# Autodesk Inventor assembly: JIMSCUBE
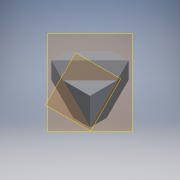
[picture p0: Inventor's stored thumbnail of the model, 180x180]
Saved by Autodesk Inventor 2019 (Build 230136000, 136)
## iProperties
Created: 2019-09-15
Part Number: JIMSCUBE
Document SubType Name: Assembly
Designer: james
Author: james
## Documents named in this file (3)
- F:\JimsDesign\P1001-16bit-CPU\P1001-001 - 16bit CPU\JIMSCUBE.iam
- F:\JimsDesign\P1001-16bit-CPU\P1001-001 - 16bit CPU\JIMSPT.ipt
- F:\JimsDesign\P1001-16bit-CPU\P1001-001 - 16bit CPU\jimscube.ipt
## Components (2 placed, 2 different names)
1. JIMSPT:1 — Mate:1, Mate:2, Mate:3
2. jimscube:1 — Mate:1, Mate:2, Mate:3
## Relationships (3: Mate 3)
- Mate:1: JIMSPT:1 ↔ jimscube:1
- Mate:2: JIMSPT:1 ↔ jimscube:1
- Mate:3: JIMSPT:1 ↔ jimscube:1
